# Autodesk Inventor assembly: sestava estonsko
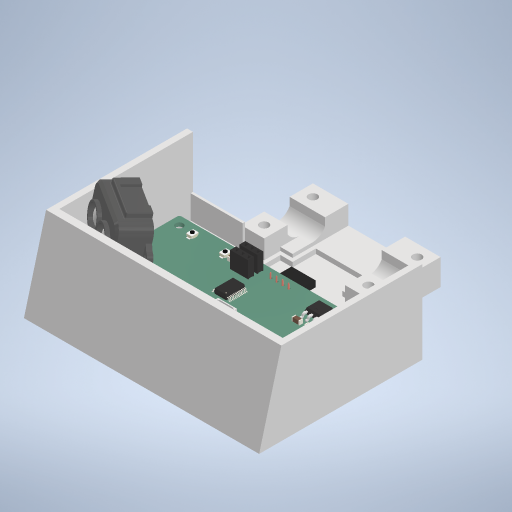
[picture p0: Inventor's stored thumbnail of the model, 512x512]
Saved by Autodesk Inventor 2024 (Build 280153000, 153)
## iProperties
Created: 2023-10-31
Part Number: sestava estonsko
Document SubType Name: Assembly
Designer: Simak
Author: Simak
## Documents named in this file (4)
- C:\Users\Simak\OneDrive\Dokumenty\GitHub\RoboCop\- 3D -\wip\sestava estonsko.iam
- C:\Users\Simak\OneDrive\Dokumenty\GitHub\RoboCop\- 3D -\el._parts\sumec\sumec.ipt
- C:\Users\Simak\OneDrive\Dokumenty\GitHub\RoboCop\- 3D -\wip\tělo estonsko.ipt
- C:\Users\Simak\OneDrive\Dokumenty\GitHub\RoboCop\sensors\TF Luna\3D\Sensor LUNA\Sensor LUNA.ipt
## Components (3 placed, 3 different names)
1. tělo estonsko:1 — Proti sobě:1, Vložit:1, Vložit:2
2. sumec:1 — Proti sobě:1, Vložit:1, Vložit:2
3. Sensor LUNA:1
## Relationships (3: Insert 2, Mate 1)
- Proti sobě:1 [Mate] (4 mm): tělo estonsko:1 ↔ sumec:1
- Vložit:1 [Insert]: tělo estonsko:1 ↔ sumec:1
- Vložit:2 [Insert]: tělo estonsko:1 ↔ sumec:1
